# Autodesk Inventor assembly: Montagem1
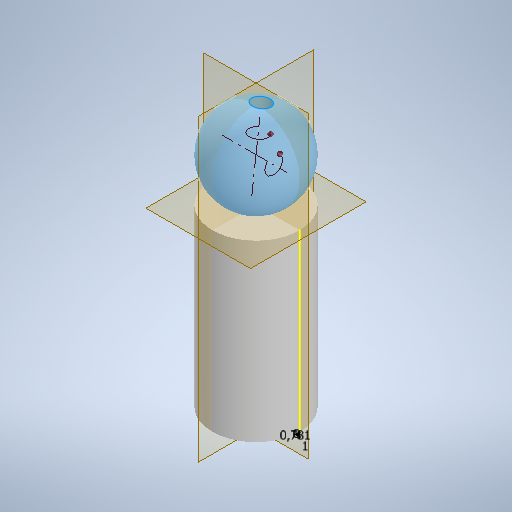
[picture p0: Inventor's stored thumbnail of the model, 512x512]
Saved by Autodesk Inventor 2025.2 (Build 292293000, 293)
## iProperties
Created: 2025-03-26
Part Number: Montagem1
Document SubType Name: Assembly
Designer: Formação
Author: Formação
## Documents named in this file (3)
- C:\Users\Formação\Documents\Inventor\Sessão_25_03_25\Montagem1.iam
- C:\Users\Formação\Documents\Inventor\Sessão_25_03_25\Peça9.ipt
- C:\Users\Formação\Documents\Inventor\Sessão_25_03_25\Peça2.1.ipt
## Components (2 placed, 2 different names)
1. Peça2.1:1 — Coincidente:4, Coincidente:6, Coincidente:7, Tangente:1, Coincidente:8, Coincidente:9
2. Peça9:1 — Coincidente:1, Coincidente:2, Coincidente:3, Coincidente:5
## Relationships (10: Mate 9, Tangent 1)
- Coincidente:1 [Mate]: Peça9:1
- Coincidente:2 [Mate]: Peça9:1
- Coincidente:3 [Mate]: Peça9:1
- Coincidente:4 [Mate]: Peça2.1:1
- Coincidente:5 [Mate]: Peça9:1
- Coincidente:6 [Mate]: Peça2.1:1
- Coincidente:7 [Mate]: Peça2.1:1
- Tangente:1 (15 mm): Peça2.1:1
- Coincidente:8 [Mate]: Peça2.1:1
- Coincidente:9 [Mate]: Peça2.1:1
